# Autodesk Inventor assembly: assembly18ghz
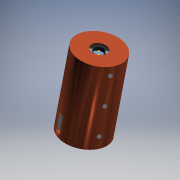
[picture p0: Inventor's stored thumbnail of the model, 180x180]
Saved by Autodesk Inventor 2017 (Build 210142000, 142)
## iProperties
Created: 2016-09-16
Part Number: assembly18ghz
Document SubType Name: Assembly
Designer: Anna
Author: Anna
## Documents named in this file (8)
- C:\Users\Anna\Documents\Inventor\Cavity2.0\Cavity final\assembly18ghz.iam
- C:\Users\Anna\Documents\Inventor\Cavity2.0\Cavity final\18ghzenclosure.ipt
- C:\Users\Anna\Documents\Inventor\Cavity2.0\Cavity final\washer.ipt
- C:\Users\Anna\Documents\Inventor\Cavity2.0\Cavity final\screw.ipt
- C:\Users\Anna\Documents\Inventor\Cavity2.0\Cavity final\Mirror.ipt
- C:\Users\Anna\Documents\Inventor\Cavity2.0\HPSt 15014-102 VS22.ipt
- C:\Users\Anna\Documents\Inventor\Cavity2.0\Cavity final\holder.ipt
- C:\Users\Anna\Documents\Inventor\Cavity2.0\Cavity final\back.ipt
## Components (10 placed, 7 different names)
1. 18ghzenclosure:1 — Mate:1, Mate:2, Mate:3, Mate:4, Mate:7, Mate:8, Mate:13, Mate:14, Mate:17, Mate:18
2. washer:1 — Mate:1, Mate:4, Mate:5
3. washer:2 — Mate:9, Mate:10, Mate:12
4. screw:1 — Mate:2, Mate:6
5. screw:2 — Mate:13, Rotational:2
6. Mirror:1 — Mate:3, Mate:5, Mate:6
7. Mirror:2 — Mate:11, Mate:12, Rotational:2
8. HPSt 15014-102 VS22:1 — Mate:8, Rotational:1, Mate:15, Mate:16
9. holder:1 — Mate:7, Rotational:1, Mate:9, Mate:10, Mate:11
10. back:1 — Mate:14, Mate:15, Mate:16, Mate:17, Mate:18
## Relationships (20: Mate 18, RevoluteJoint 2)
- Mate:1: 18ghzenclosure:1 ↔ washer:1
- Mate:2: 18ghzenclosure:1 ↔ screw:1
- Mate:3: 18ghzenclosure:1 ↔ Mirror:1
- Mate:4: 18ghzenclosure:1 ↔ washer:1
- Mate:5: washer:1 ↔ Mirror:1
- Mate:6: screw:1 ↔ Mirror:1
- Mate:7: 18ghzenclosure:1 ↔ holder:1
- Mate:8: 18ghzenclosure:1 ↔ HPSt 15014-102 VS22:1
- Rotational:1 [RevoluteJoint]: HPSt 15014-102 VS22:1 ↔ holder:1
- Mate:9: washer:2 ↔ holder:1
- Mate:10: washer:2 ↔ holder:1
- Mate:11: Mirror:2 ↔ holder:1
- Mate:12: washer:2 ↔ Mirror:2
- Mate:13: 18ghzenclosure:1 ↔ screw:2
- Rotational:2 [RevoluteJoint]: screw:2 ↔ Mirror:2
- Mate:14: 18ghzenclosure:1 ↔ back:1
- Mate:15: HPSt 15014-102 VS22:1 ↔ back:1
- Mate:16: HPSt 15014-102 VS22:1 ↔ back:1
- Mate:17: 18ghzenclosure:1 ↔ back:1
- Mate:18: 18ghzenclosure:1 ↔ back:1
